# Autodesk Inventor assembly: Corpo1
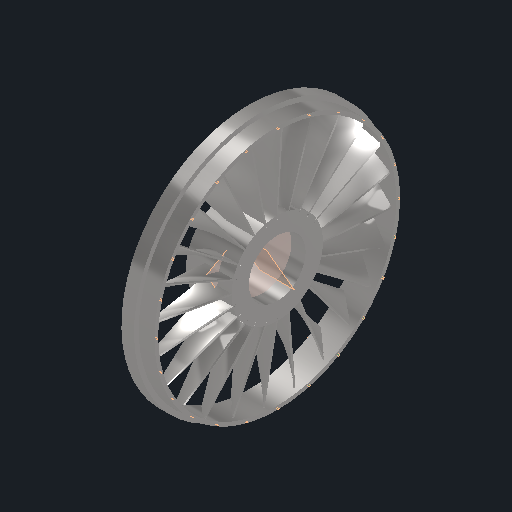
[picture p0: Inventor's stored thumbnail of the model, 512x512]
Saved by Autodesk Inventor 2026.2 (Build 302298010, 298A)
## iProperties
Created: 2026-05-01
Part Number: Corpo1
Document SubType Name: Assembly
Designer: Yan
Author: Yan
## Documents named in this file (4)
- C:\Users\Yan\Desktop\Turbina\Corpo1.iam
- C:\Users\Yan\Desktop\Turbina\PalaCorpoStadio1.ipt
- C:\Users\Yan\Desktop\Turbina\CorpoDiscoPaleSatdio1-DimensioniAprossimate.ipt
- C:\Users\Yan\Desktop\Turbina\DiscoCorpoTurbina1.ipt
## Components (26 placed, 3 different names)
1. PalaCorpoStadio1:1 — Mate:7, Mate:43, Flush:17
2. PalaCorpoStadio1:2 — Mate:2, Mate:48, Flush:22
3. PalaCorpoStadio1:3 — Mate:8, Mate:42, Flush:16
4. PalaCorpoStadio1:4 — Mate:9, Mate:41, Flush:15
5. PalaCorpoStadio1:5 — Mate:1, Mate:32, Flush:23
6. PalaCorpoStadio1:6 — Mate:14, Mate:36, Flush:10
7. PalaCorpoStadio1:7 — Mate:10, Mate:40, Flush:14
8. PalaCorpoStadio1:8 — Mate:16, Mate:34, Flush:8
9. PalaCorpoStadio1:9 — Mate:11, Mate:39, Flush:13
10. PalaCorpoStadio1:10 — Mate:15, Mate:35, Flush:9
11. PalaCorpoStadio1:11 — Mate:12, Mate:38, Flush:12
12. PalaCorpoStadio1:12 — Mate:13, Mate:37, Flush:11
13. PalaCorpoStadio1:13 — Mate:3, Mate:47, Flush:21
14. PalaCorpoStadio1:14 — Mate:6, Mate:44, Flush:18
15. PalaCorpoStadio1:15 — Mate:19, Mate:26, Flush:5
16. PalaCorpoStadio1:16 — Mate:20, Mate:25, Flush:4
17. PalaCorpoStadio1:17 — Mate:18, Mate:27, Flush:6
18. PalaCorpoStadio1:18 — Mate:17, Mate:33, Flush:7
19. PalaCorpoStadio1:19 — Mate:4, Mate:46, Flush:20
20. PalaCorpoStadio1:20 — Mate:5, Mate:45, Flush:19
21. PalaCorpoStadio1:21 — Mate:28, Mate:30, Flush:1
22. PalaCorpoStadio1:22 — Mate:29, Mate:31, Flush:24
23. PalaCorpoStadio1:23 — Mate:22, Mate:23, Flush:2
24. PalaCorpoStadio1:24 — Mate:21, Mate:24, Flush:3
25. CorpoDiscoPaleSatdio1-DimensioniAprossimate:1 — Mate:1, Mate:2, Mate:3, Mate:4, Mate:5, Mate:6, Mate:7, Mate:8, Mate:9, Mate:10, Mate:11, Mate:12, Mate:13, Mate:14, Mate:15, Mate:16, Mate:17, Mate:18, Mate:19, Mate:20, Mate:21, Mate:22, Mate:23, Mate:24, Mate:25, Mate:26, Mate:27, Mate:28, Mate:29, Mate:30, Mate:31, Mate:32, Mate:33, Mate:34, Mate:35, Mate:36, Mate:37, Mate:38, Mate:39, Mate:40, Mate:41, Mate:42, Mate:43, Mate:44, Mate:45, Mate:46, Mate:47, Mate:48, Flush:1, Flush:2, Flush:3, Flush:4, Flush:5, Flush:6, Flush:7, Flush:8, Flush:9, Flush:10, Flush:11, Flush:12, Flush:13, Flush:14, Flush:15, Flush:16, Flush:17, Flush:18, Flush:19, Flush:20, Flush:21, Flush:22, Flush:23, Flush:24, Mate:49, Flush:25
26. DiscoCorpoTurbina1:1 — Mate:49, Flush:25
## Relationships (74: Mate 49, Flush 25)
- Mate:1: PalaCorpoStadio1:5 ↔ CorpoDiscoPaleSatdio1-DimensioniAprossimate:1
- Mate:2: PalaCorpoStadio1:2 ↔ CorpoDiscoPaleSatdio1-DimensioniAprossimate:1
- Mate:3: PalaCorpoStadio1:13 ↔ CorpoDiscoPaleSatdio1-DimensioniAprossimate:1
- Mate:4: PalaCorpoStadio1:19 ↔ CorpoDiscoPaleSatdio1-DimensioniAprossimate:1
- Mate:5: PalaCorpoStadio1:20 ↔ CorpoDiscoPaleSatdio1-DimensioniAprossimate:1
- Mate:6: PalaCorpoStadio1:14 ↔ CorpoDiscoPaleSatdio1-DimensioniAprossimate:1
- Mate:7: PalaCorpoStadio1:1 ↔ CorpoDiscoPaleSatdio1-DimensioniAprossimate:1
- Mate:8: PalaCorpoStadio1:3 ↔ CorpoDiscoPaleSatdio1-DimensioniAprossimate:1
- Mate:9: PalaCorpoStadio1:4 ↔ CorpoDiscoPaleSatdio1-DimensioniAprossimate:1
- Mate:10: PalaCorpoStadio1:7 ↔ CorpoDiscoPaleSatdio1-DimensioniAprossimate:1
- Mate:11: PalaCorpoStadio1:9 ↔ CorpoDiscoPaleSatdio1-DimensioniAprossimate:1
- Mate:12: PalaCorpoStadio1:11 ↔ CorpoDiscoPaleSatdio1-DimensioniAprossimate:1
- Mate:13: PalaCorpoStadio1:12 ↔ CorpoDiscoPaleSatdio1-DimensioniAprossimate:1
- Mate:14: PalaCorpoStadio1:6 ↔ CorpoDiscoPaleSatdio1-DimensioniAprossimate:1
- Mate:15: PalaCorpoStadio1:10 ↔ CorpoDiscoPaleSatdio1-DimensioniAprossimate:1
- Mate:16: PalaCorpoStadio1:8 ↔ CorpoDiscoPaleSatdio1-DimensioniAprossimate:1
- Mate:17: PalaCorpoStadio1:18 ↔ CorpoDiscoPaleSatdio1-DimensioniAprossimate:1
- Mate:18: PalaCorpoStadio1:17 ↔ CorpoDiscoPaleSatdio1-DimensioniAprossimate:1
- Mate:19: PalaCorpoStadio1:15 ↔ CorpoDiscoPaleSatdio1-DimensioniAprossimate:1
- Mate:20: PalaCorpoStadio1:16 ↔ CorpoDiscoPaleSatdio1-DimensioniAprossimate:1
- Mate:21: PalaCorpoStadio1:24 ↔ CorpoDiscoPaleSatdio1-DimensioniAprossimate:1
- Mate:22: PalaCorpoStadio1:23 ↔ CorpoDiscoPaleSatdio1-DimensioniAprossimate:1
- Mate:23: PalaCorpoStadio1:23 ↔ CorpoDiscoPaleSatdio1-DimensioniAprossimate:1
- Mate:24: PalaCorpoStadio1:24 ↔ CorpoDiscoPaleSatdio1-DimensioniAprossimate:1
- Mate:25: PalaCorpoStadio1:16 ↔ CorpoDiscoPaleSatdio1-DimensioniAprossimate:1
- Mate:26: PalaCorpoStadio1:15 ↔ CorpoDiscoPaleSatdio1-DimensioniAprossimate:1
- Mate:27: PalaCorpoStadio1:17 ↔ CorpoDiscoPaleSatdio1-DimensioniAprossimate:1
- Mate:28: PalaCorpoStadio1:21 ↔ CorpoDiscoPaleSatdio1-DimensioniAprossimate:1
- Mate:29: PalaCorpoStadio1:22 ↔ CorpoDiscoPaleSatdio1-DimensioniAprossimate:1
- Mate:30: PalaCorpoStadio1:21 ↔ CorpoDiscoPaleSatdio1-DimensioniAprossimate:1
- Mate:31: PalaCorpoStadio1:22 ↔ CorpoDiscoPaleSatdio1-DimensioniAprossimate:1
- Mate:32: PalaCorpoStadio1:5 ↔ CorpoDiscoPaleSatdio1-DimensioniAprossimate:1
- Mate:33: PalaCorpoStadio1:18 ↔ CorpoDiscoPaleSatdio1-DimensioniAprossimate:1
- Mate:34: PalaCorpoStadio1:8 ↔ CorpoDiscoPaleSatdio1-DimensioniAprossimate:1
- Mate:35: PalaCorpoStadio1:10 ↔ CorpoDiscoPaleSatdio1-DimensioniAprossimate:1
- Mate:36: PalaCorpoStadio1:6 ↔ CorpoDiscoPaleSatdio1-DimensioniAprossimate:1
- Mate:37: PalaCorpoStadio1:12 ↔ CorpoDiscoPaleSatdio1-DimensioniAprossimate:1
- Mate:38: PalaCorpoStadio1:11 ↔ CorpoDiscoPaleSatdio1-DimensioniAprossimate:1
- Mate:39: PalaCorpoStadio1:9 ↔ CorpoDiscoPaleSatdio1-DimensioniAprossimate:1
- Mate:40: PalaCorpoStadio1:7 ↔ CorpoDiscoPaleSatdio1-DimensioniAprossimate:1
- Mate:41: PalaCorpoStadio1:4 ↔ CorpoDiscoPaleSatdio1-DimensioniAprossimate:1
- Mate:42: PalaCorpoStadio1:3 ↔ CorpoDiscoPaleSatdio1-DimensioniAprossimate:1
- Mate:43: PalaCorpoStadio1:1 ↔ CorpoDiscoPaleSatdio1-DimensioniAprossimate:1
- Mate:44: PalaCorpoStadio1:14 ↔ CorpoDiscoPaleSatdio1-DimensioniAprossimate:1
- Mate:45: PalaCorpoStadio1:20 ↔ CorpoDiscoPaleSatdio1-DimensioniAprossimate:1
- Mate:46: PalaCorpoStadio1:19 ↔ CorpoDiscoPaleSatdio1-DimensioniAprossimate:1
- Mate:47: PalaCorpoStadio1:13 ↔ CorpoDiscoPaleSatdio1-DimensioniAprossimate:1
- Mate:48: PalaCorpoStadio1:2 ↔ CorpoDiscoPaleSatdio1-DimensioniAprossimate:1
- Flush:1: PalaCorpoStadio1:21 ↔ CorpoDiscoPaleSatdio1-DimensioniAprossimate:1
- Flush:2: PalaCorpoStadio1:23 ↔ CorpoDiscoPaleSatdio1-DimensioniAprossimate:1
- Flush:3: PalaCorpoStadio1:24 ↔ CorpoDiscoPaleSatdio1-DimensioniAprossimate:1
- Flush:4: PalaCorpoStadio1:16 ↔ CorpoDiscoPaleSatdio1-DimensioniAprossimate:1
- Flush:5: PalaCorpoStadio1:15 ↔ CorpoDiscoPaleSatdio1-DimensioniAprossimate:1
- Flush:6: PalaCorpoStadio1:17 ↔ CorpoDiscoPaleSatdio1-DimensioniAprossimate:1
- Flush:7: PalaCorpoStadio1:18 ↔ CorpoDiscoPaleSatdio1-DimensioniAprossimate:1
- Flush:8: PalaCorpoStadio1:8 ↔ CorpoDiscoPaleSatdio1-DimensioniAprossimate:1
- Flush:9: PalaCorpoStadio1:10 ↔ CorpoDiscoPaleSatdio1-DimensioniAprossimate:1
- Flush:10: PalaCorpoStadio1:6 ↔ CorpoDiscoPaleSatdio1-DimensioniAprossimate:1
- Flush:11: PalaCorpoStadio1:12 ↔ CorpoDiscoPaleSatdio1-DimensioniAprossimate:1
- Flush:12: PalaCorpoStadio1:11 ↔ CorpoDiscoPaleSatdio1-DimensioniAprossimate:1
- Flush:13: PalaCorpoStadio1:9 ↔ CorpoDiscoPaleSatdio1-DimensioniAprossimate:1
- Flush:14: PalaCorpoStadio1:7 ↔ CorpoDiscoPaleSatdio1-DimensioniAprossimate:1
- Flush:15: PalaCorpoStadio1:4 ↔ CorpoDiscoPaleSatdio1-DimensioniAprossimate:1
- Flush:16: PalaCorpoStadio1:3 ↔ CorpoDiscoPaleSatdio1-DimensioniAprossimate:1
- Flush:17: PalaCorpoStadio1:1 ↔ CorpoDiscoPaleSatdio1-DimensioniAprossimate:1
- Flush:18: PalaCorpoStadio1:14 ↔ CorpoDiscoPaleSatdio1-DimensioniAprossimate:1
- Flush:19: PalaCorpoStadio1:20 ↔ CorpoDiscoPaleSatdio1-DimensioniAprossimate:1
- Flush:20: PalaCorpoStadio1:19 ↔ CorpoDiscoPaleSatdio1-DimensioniAprossimate:1
- Flush:21: PalaCorpoStadio1:13 ↔ CorpoDiscoPaleSatdio1-DimensioniAprossimate:1
- Flush:22: PalaCorpoStadio1:2 ↔ CorpoDiscoPaleSatdio1-DimensioniAprossimate:1
- Flush:23: PalaCorpoStadio1:5 ↔ CorpoDiscoPaleSatdio1-DimensioniAprossimate:1
- Flush:24: PalaCorpoStadio1:22 ↔ CorpoDiscoPaleSatdio1-DimensioniAprossimate:1
- Mate:49: CorpoDiscoPaleSatdio1-DimensioniAprossimate:1 ↔ DiscoCorpoTurbina1:1
- Flush:25: CorpoDiscoPaleSatdio1-DimensioniAprossimate:1 ↔ DiscoCorpoTurbina1:1
